# Autodesk Inventor assembly: !Crossbrace
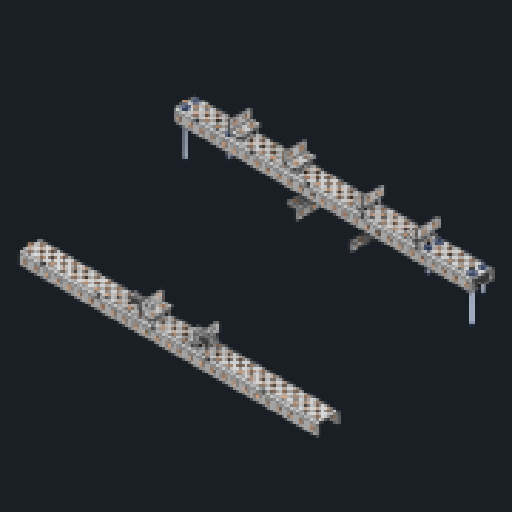
[picture p0: Inventor's stored thumbnail of the model, 512x512]
Saved by Autodesk Inventor 2025 (Build 290162000, 162)
## iProperties
Created: 2024-12-18
Part Number: !Crossbrace
Document SubType Name: Assembly
Designer: avere
Author: avere
## Documents named in this file (18)
- D:\VEX\High Stakes\CAD\V4\Chassis\Crossbrace\!Crossbrace.iam
- D:\VEX\High Stakes\CAD\ROBOPROS-CAD-Inventor\Structure\C Channel\Aluminum 1x2x1\Alu C 1x2x1x27.ipt
- D:\VEX\High Stakes\CAD\ROBOPROS-CAD-Inventor\Motion\Spacers\Spacer Nylon .375 OD\NSpacer .375 OD x .500.ipt
- D:\VEX\High Stakes\CAD\ROBOPROS-CAD-Inventor\Motion\Spacers\Spacer Nylon .375 OD.ipt
- D:\VEX\High Stakes\CAD\ROBOPROS-CAD-Inventor\Structure\Hardware\Screw Shoulder Robosource\SScrew Shoulder Smooth 2.000 x .04.ipt
- D:\VEX\High Stakes\CAD\ROBOPROS-CAD-Inventor\Structure\Hardware\Screw Shoulder Robosource.ipt
- D:\VEX\High Stakes\CAD\ROBOPROS-CAD-Inventor\Structure\Hardware\Screw Steel - Star\SScrew Star Smooth 1.000.ipt
- D:\VEX\High Stakes\CAD\ROBOPROS-CAD-Inventor\Structure\Hardware\Screw Steel - Star.ipt
- D:\VEX\High Stakes\CAD\ROBOPROS-CAD-Inventor\Modified Parts\Bearing Flat Low Profile 2-Hole.ipt
- D:\VEX\High Stakes\CAD\ROBOPROS-CAD-Inventor\Structure\Angle\Aluminum 1x1\Alu Angle 1x1x2.ipt
- D:\VEX\High Stakes\CAD\ROBOPROS-CAD-Inventor\Structure\1-Post Standoff Retainer.ipt
- D:\VEX\High Stakes\CAD\ROBOPROS-CAD-Inventor\Structure\Standoff\Standoff .25.ipt
- D:\VEX\High Stakes\CAD\ROBOPROS-CAD-Inventor\Structure\Standoff.ipt
- D:\VEX\High Stakes\CAD\ROBOPROS-CAD-Inventor\Structure\1-Post Hex Nut Retainer With Hardware.iam
- D:\VEX\High Stakes\CAD\ROBOPROS-CAD-Inventor\Motion\Spacers\Spacer Nylon .375 OD\NSpacer .375 OD x .375.ipt
- D:\VEX\High Stakes\CAD\ROBOPROS-CAD-Inventor\Motion\Spacers\Washer Steel\SWasher .375 OD x .015625.ipt
- D:\VEX\High Stakes\CAD\ROBOPROS-CAD-Inventor\Motion\Spacers\Washer Steel.ipt
- D:\VEX\High Stakes\CAD\ROBOPROS-CAD-Inventor\Motion\Spacers\Washer Steel\SWasher .375 OD x .062500.ipt
## Components (46 placed, 12 different names)
1. Alu C 1x2x1x27:1 — Mate:1, Flush:1, Flush:2, Mate:2, Mate:3, Flush:3, Insert:20, Mate:4, Insert:32, Mate:16
2. Alu C 1x2x1x27:2 — Mate:2, Mate:3, Flush:3, Insert:1, Insert:2, Insert:3, Insert:4, Insert:5, Insert:6, Insert:7, Insert:8, Insert:9, Insert:11, Insert:14, Insert:15, Insert:16, Insert:17, Insert:18, Insert:19, Insert:27, Mate:11, Insert:29, Mate:13, Insert:34, Mate:18, Insert:36, Mate:20, Insert:37, Mate:21, Insert:38, Mate:22
3. NSpacer .375 OD x .500:1 — Insert:4
4. NSpacer .375 OD x .500:2 — Insert:3
5. NSpacer .375 OD x .500:3 — Insert:2
6. NSpacer .375 OD x .500:4 — Insert:1
7. NSpacer .375 OD x .500:5 — Insert:6
8. NSpacer .375 OD x .500:6 — Insert:5
9. NSpacer .375 OD x .500:7 — Insert:8
10. NSpacer .375 OD x .500:8 — Insert:7
11. SScrew Shoulder Smooth 2.000 x .04:2 — Insert:9
12. SScrew Shoulder Smooth 2.000 x .04:4 — Insert:11
13. SScrew Star Smooth 1.000:1 — Insert:15
14. SScrew Star Smooth 1.000:2 — Insert:14
15. SScrew Star Smooth 1.000:3 — Insert:16
16. SScrew Star Smooth 1.000:4 — Insert:17
17. SScrew Star Smooth 1.000:5 — Insert:18
18. SScrew Star Smooth 1.000:6 — Insert:19
19. Bearing Flat Low Profile 2-Hole:1 — Insert:31, Mate:15, Insert:32, Mate:16
20. Bearing Flat Low Profile 2-Hole:2 — Insert:20, Mate:4, Insert:30, Mate:14
21. Alu Angle 1x1x2:1 — Insert:30, Mate:14, Insert:43, Mate:24, Insert:56
22. Alu Angle 1x1x2:2 — Insert:31, Mate:15, Insert:44, Mate:25, Insert:55
23. Bearing Flat Low Profile 2-Hole:3 — Insert:27, Mate:23
24. Alu Angle 1x1x2:3 — Mate:11, Mate:23
25. Bearing Flat Low Profile 2-Hole:4 — Insert:29
26. Alu Angle 1x1x2:4 — Mate:13
27. Bearing Flat Low Profile 2-Hole:5 — Insert:34
28. Alu Angle 1x1x2:5 — Mate:18, Insert:50, Mate:27
29. Bearing Flat Low Profile 2-Hole:6 — Insert:36
30. Alu Angle 1x1x2:6 — Mate:20, Insert:47, Mate:26
31. Alu Angle 1x1x2:7 — Insert:37, Mate:21
32. Alu Angle 1x1x2:8 — Insert:38, Mate:22
33. 1-Post Standoff Retainer:1 — Insert:43, Mate:24, Insert:45, Angle:1
34. 1-Post Standoff Retainer:2 — Insert:44, Mate:25, Insert:46, Angle:2
35. Standoff .25:1 — Insert:45, Angle:1
36. Standoff .25:2 — Insert:46, Angle:2
37. NSpacer .375 OD x .500:11 — Insert:47, Insert:48
38. 1-Post Hex Nut Retainer With Hardware:1 [sub-assembly] — Insert:48, Mate:26
39. NSpacer .375 OD x .500:12 — Insert:50
40. 1-Post Hex Nut Retainer With Hardware:2 [sub-assembly] — Mate:27
41. NSpacer .375 OD x .375:13 — Insert:51, Insert:56
42. SWasher .375 OD x .015625:1 — Insert:52
43. SWasher .375 OD x .062500:2 — Insert:51, Insert:52
44. NSpacer .375 OD x .375:14 — Insert:55
45. SWasher .375 OD x .015625:3
46. SWasher .375 OD x .062500:4
## Relationships (70: Insert 43, Mate 22, Flush 3, Angle 2)
- Mate:1 (76.2 mm): Alu C 1x2x1x27:1
- Flush:1 (-171.45 mm): Alu C 1x2x1x27:1
- Flush:2 (-17.4625 mm): Alu C 1x2x1x27:1
- Mate:2 (39.6875 mm): Alu C 1x2x1x27:1 ↔ Alu C 1x2x1x27:2
- Mate:3 (152.4 mm): Alu C 1x2x1x27:1 ↔ Alu C 1x2x1x27:2
- Flush:3: Alu C 1x2x1x27:1 ↔ Alu C 1x2x1x27:2
- Insert:1: Alu C 1x2x1x27:2 ↔ NSpacer .375 OD x .500:4
- Insert:2: Alu C 1x2x1x27:2 ↔ NSpacer .375 OD x .500:3
- Insert:3: Alu C 1x2x1x27:2 ↔ NSpacer .375 OD x .500:2
- Insert:4: Alu C 1x2x1x27:2 ↔ NSpacer .375 OD x .500:1
- Insert:5: Alu C 1x2x1x27:2 ↔ NSpacer .375 OD x .500:6
- Insert:6: Alu C 1x2x1x27:2 ↔ NSpacer .375 OD x .500:5
- Insert:7: Alu C 1x2x1x27:2 ↔ NSpacer .375 OD x .500:8
- Insert:8: Alu C 1x2x1x27:2 ↔ NSpacer .375 OD x .500:7
- Insert:9: Alu C 1x2x1x27:2 ↔ SScrew Shoulder Smooth 2.000 x .04:2
- Insert:11: Alu C 1x2x1x27:2 ↔ SScrew Shoulder Smooth 2.000 x .04:4
- Insert:14: Alu C 1x2x1x27:2 ↔ SScrew Star Smooth 1.000:2
- Insert:15: Alu C 1x2x1x27:2 ↔ SScrew Star Smooth 1.000:1
- Insert:16: Alu C 1x2x1x27:2 ↔ SScrew Star Smooth 1.000:3
- Insert:17: Alu C 1x2x1x27:2 ↔ SScrew Star Smooth 1.000:4
- Insert:18: Alu C 1x2x1x27:2 ↔ SScrew Star Smooth 1.000:5
- Insert:19: Alu C 1x2x1x27:2 ↔ SScrew Star Smooth 1.000:6
- Insert:20: Alu C 1x2x1x27:1 ↔ Bearing Flat Low Profile 2-Hole:2
- Mate:4: Alu C 1x2x1x27:1 ↔ Bearing Flat Low Profile 2-Hole:2
- [Mate]: Bearing Flat Low Profile 2-Hole:3 ↔ Alu Angle 1x1x2:3
- Insert:27: Alu C 1x2x1x27:2 ↔ Bearing Flat Low Profile 2-Hole:3
- Mate:11: Alu C 1x2x1x27:2 ↔ Alu Angle 1x1x2:3
- [Insert] (1.27 mm): Bearing Flat Low Profile 2-Hole:4 ↔ Alu Angle 1x1x2:4
- [Mate]: Bearing Flat Low Profile 2-Hole:4 ↔ Alu Angle 1x1x2:4
- Insert:29: Alu C 1x2x1x27:2 ↔ Bearing Flat Low Profile 2-Hole:4
- Mate:13: Alu C 1x2x1x27:2 ↔ Alu Angle 1x1x2:4
- Insert:30 (1.27 mm): Bearing Flat Low Profile 2-Hole:2 ↔ Alu Angle 1x1x2:1
- Mate:14: Bearing Flat Low Profile 2-Hole:2 ↔ Alu Angle 1x1x2:1
- Insert:31 (1.27 mm): Bearing Flat Low Profile 2-Hole:1 ↔ Alu Angle 1x1x2:2
- Mate:15: Bearing Flat Low Profile 2-Hole:1 ↔ Alu Angle 1x1x2:2
- Insert:32: Alu C 1x2x1x27:1 ↔ Bearing Flat Low Profile 2-Hole:1
- Mate:16: Alu C 1x2x1x27:1 ↔ Bearing Flat Low Profile 2-Hole:1
- [Insert] (1.27 mm): Bearing Flat Low Profile 2-Hole:5 ↔ Alu Angle 1x1x2:5
- [Mate]: Bearing Flat Low Profile 2-Hole:5 ↔ Alu Angle 1x1x2:5
- Insert:34: Alu C 1x2x1x27:2 ↔ Bearing Flat Low Profile 2-Hole:5
- Mate:18: Alu C 1x2x1x27:2 ↔ Alu Angle 1x1x2:5
- [Insert] (1.27 mm): Bearing Flat Low Profile 2-Hole:6 ↔ Alu Angle 1x1x2:6
- [Mate]: Bearing Flat Low Profile 2-Hole:6 ↔ Alu Angle 1x1x2:6
- Insert:36: Alu C 1x2x1x27:2 ↔ Bearing Flat Low Profile 2-Hole:6
- Mate:20: Alu C 1x2x1x27:2 ↔ Alu Angle 1x1x2:6
- Insert:37 (28.575 mm): Alu C 1x2x1x27:2 ↔ Alu Angle 1x1x2:7
- Mate:21: Alu C 1x2x1x27:2 ↔ Alu Angle 1x1x2:7
- Insert:38 (28.575 mm): Alu C 1x2x1x27:2 ↔ Alu Angle 1x1x2:8
- Mate:22: Alu C 1x2x1x27:2 ↔ Alu Angle 1x1x2:8
- Mate:23: Bearing Flat Low Profile 2-Hole:3 ↔ Alu Angle 1x1x2:3
- Insert:43: Alu Angle 1x1x2:1 ↔ 1-Post Standoff Retainer:1
- Mate:24: Alu Angle 1x1x2:1 ↔ 1-Post Standoff Retainer:1
- Insert:44: Alu Angle 1x1x2:2 ↔ 1-Post Standoff Retainer:2
- Mate:25: Alu Angle 1x1x2:2 ↔ 1-Post Standoff Retainer:2
- Insert:45: 1-Post Standoff Retainer:1 ↔ Standoff .25:1
- Angle:1 (0 deg): 1-Post Standoff Retainer:1 ↔ Standoff .25:1
- Insert:46: 1-Post Standoff Retainer:2 ↔ Standoff .25:2
- Angle:2 (0 deg): 1-Post Standoff Retainer:2 ↔ Standoff .25:2
- Insert:47: Alu Angle 1x1x2:6 ↔ NSpacer .375 OD x .500:11
- Insert:48 (1.5875 mm): NSpacer .375 OD x .500:11 ↔ 1-Post Hex Nut Retainer With Hardware:1
- Mate:26: Alu Angle 1x1x2:6 ↔ 1-Post Hex Nut Retainer With Hardware:1
- [Insert] (1.5875 mm): NSpacer .375 OD x .500:12 ↔ 1-Post Hex Nut Retainer With Hardware:2
- Insert:50: Alu Angle 1x1x2:5 ↔ NSpacer .375 OD x .500:12
- Mate:27: Alu Angle 1x1x2:5 ↔ 1-Post Hex Nut Retainer With Hardware:2
- Insert:51: NSpacer .375 OD x .375:13 ↔ SWasher .375 OD x .062500:2
- Insert:52: SWasher .375 OD x .015625:1 ↔ SWasher .375 OD x .062500:2
- [Insert]: NSpacer .375 OD x .375:14 ↔ SWasher .375 OD x .062500:4
- [Insert]: SWasher .375 OD x .015625:3 ↔ SWasher .375 OD x .062500:4
- Insert:55: Alu Angle 1x1x2:2 ↔ NSpacer .375 OD x .375:14
- Insert:56: Alu Angle 1x1x2:1 ↔ NSpacer .375 OD x .375:13
## Named parameters: d39_d37 = 0 mm, d42_d38_d36 = 1.27 mm, d43_d39_d37 = 0 mm, d54_d38_d36 = 1.27 mm, d55_d39_d37 = 0 mm, d58_d38_d36 = 1.27 mm, d59_d39_d37 = 0 mm, d84_d82 = 1.5875 mm, d89_d87 = 0 mm, d90_d88 = 0 mm
